# Autodesk Inventor assembly: Assembly_Planktoscope_Lid_Screen
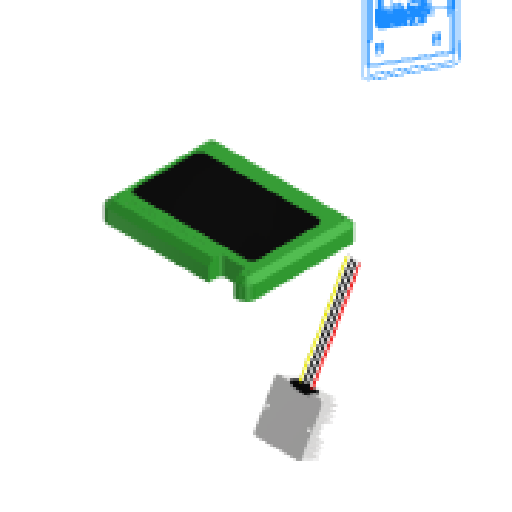
[picture p0: Inventor's stored thumbnail of the model, 512x512]
Saved by Autodesk Inventor 2025.1 (Build 291241020, 241B)
## iProperties
Created: 2024-06-29
Part Number: Assembly_Planktoscope_Lid_Screen
Document SubType Name: Assembly
Designer: diederichbenedict
Mass: 1274.9 g
Surface Area: 4345.43 cm^2
Volume: 1274.9 cm^3
Density: 1 g/cm^3
Author: diederichbenedict
## Documents named in this file (5)
- C:\Users\diederichbenedict\Dropbox\Dokumente\Promotion\PROJECTS\openUC2_SOOP\INVENTOR\Workspace\Assembly_Planktoscope_Lid_Screen.iam
- C:\Users\diederichbenedict\Dropbox\Dokumente\Promotion\PROJECTS\openUC2_SOOP\INVENTOR\Workspace\00_raspberry pi display\00_raspberry pi display.ipt
- C:\Users\diederichbenedict\Dropbox\Dokumente\Promotion\PROJECTS\openUC2_SOOP\INVENTOR\Workspace\00_OutdoorCase_Type2000_toplid.ipt
- C:\Users\diederichbenedict\Dropbox\Dokumente\Promotion\PROJECTS\openUC2_SOOP\INVENTOR\Workspace\60_Planktoscope_RaspiScreenHolder_v0.ipt
- C:\Users\diederichbenedict\Dropbox\Dokumente\Promotion\PROJECTS\openUC2_SOOP\INVENTOR\Workspace\00_360W_DCDCCONVERTER_12V-5V_10A\00_360W_DCDCCONVERTER_12V-5V_10A.ipt
## Components (4 placed, 4 different names)
1. 00_raspberry pi display:1 — Mate:1, Mate:2, Mate:3
2. 00_OutdoorCase_Type2000_toplid:1 — Mate:1, Mate:2, Mate:3, Flush:1, Flush:2
3. 00_360W_DCDCCONVERTER_12V-5V_10A:1
4. 60_Planktoscope_RaspiScreenHolder_v0:1 — Flush:1, Flush:2
## Relationships (5: Mate 3, Flush 2)
- Mate:1: 00_raspberry pi display:1 ↔ 00_OutdoorCase_Type2000_toplid:1
- Mate:2 (5 mm): 00_raspberry pi display:1 ↔ 00_OutdoorCase_Type2000_toplid:1
- Mate:3 (5 mm): 00_raspberry pi display:1 ↔ 00_OutdoorCase_Type2000_toplid:1
- Flush:1: 00_OutdoorCase_Type2000_toplid:1 ↔ 60_Planktoscope_RaspiScreenHolder_v0:1
- Flush:2: 00_OutdoorCase_Type2000_toplid:1 ↔ 60_Planktoscope_RaspiScreenHolder_v0:1
